# Autodesk Inventor assembly: turret_assembly
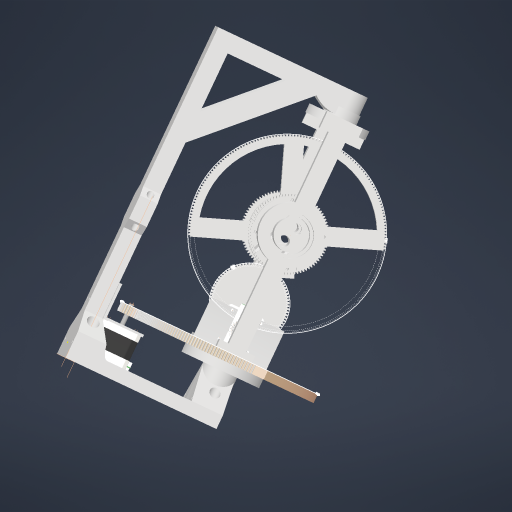
[picture p0: Inventor's stored thumbnail of the model, 512x512]
Saved by Autodesk Inventor 2023.2 (Build 272271000, 271)
## iProperties
Created: 2020-09-03
Part Number: turret_assembly
Document SubType Name: Assembly
Designer: bober
Author: bober
## Documents named in this file (19)
- F:\Turret\Our\Models\turret_assembly.iam
- F:\Turret\Our\Models\turret_assembly\Design Accelerator\vertical_axis_small_gear.ipt
- F:\Turret\Our\Models\turret_assembly\Design Accelerator\vertical_axis_bigl_gear.ipt
- F:\Turret\Our\Models\turret_assembly\Design Accelerator\horizontal_axis_big_gear.ipt
- F:\Turret\Our\Models\turret_assembly\Design Accelerator\pylon.ipt
- F:\Turret\Our\Models\turret_assembly\Design Accelerator\upper_grip.ipt
- F:\Turret\Our\Models\turret_assembly\Design Accelerator\main_stand_lower_half.ipt
- F:\Turret\Our\Models\turret_assembly\Design Accelerator\main_stand_upper_half.ipt
- F:\Turret\Our\Models\step_motor\Nema 17 Motor a Pasos 17HS4401.iam
- F:\Turret\Our\Models\turret_assembly\Design Accelerator\horizontal_lower_bearing_holder.ipt
- F:\Turret\Our\Models\turret_assembly\Design Accelerator\horizontal_axis_motor_metal_holder.ipt
- F:\Turret\Our\Models\turret_assembly\Design Accelerator\vertical_axis_motor_metal_holder.ipt
- F:\Turret\Our\Models\turret_assembly\Design Accelerator\Swash_distance.ipt
- F:\Turret\Our\Models\turret_assembly\Design Accelerator\big_actuator_holder.ipt
- F:\Turret\Our\Models\pylon_actuator_holder.ipt
- F:\Turret\Our\Models\pylon_actuator_holder_jaw.ipt
- F:\Turret\Our\Models\vertical_axis_hal_holder.ipt
- F:\Turret\Our\Models\turret_assembly\Design Accelerator\Spur Gears1.iam
- F:\Turret\Our\Models\turret_assembly\Design Accelerator\horizontal_axis_hal_gearr.ipt
## Components (23 placed, 18 different names)
1. vertical_axis_small_gear:1 — Tangent:1, Mate:4, Flush:1
2. horizontal_axis_big_gear:1 — Rigid:19, Insert:10
3. vertical_axis_small_gear:2 — Rotational:14
4. vertical_axis_bigl_gear:2 — Rigid:11, Rigid:12, Rigid:20, Rigid:21, Tangent:1, Flush:1
5. pylon:1 — Rigid:21, Flush:2, Insert:1
6. pylon:2 — Rigid:20, Rigid:22, Insert:4
7. upper_grip:1 — Rigid:22, Flush:3, Insert:11, Insert:12
8. main_stand_lower_half:1 — Rigid:5, Rotational:12, Mate:1, Mate:2, Rigid:15, Mate:3
9. main_stand_upper_half:1 — Rigid:15
10. Nema 17 Motor a Pasos 17HS4401:2 [sub-assembly] — Mate:3, Mate:4
11. Nema 17 Motor a Pasos 17HS4401:3 [sub-assembly] — Rigid:13, Rotational:14
12. horizontal_lower_bearing_holder:1 — Rigid:11, Rotational:11
13. horizontal_axis_motor_metal_holder:1 — Rigid:12, Rigid:13
14. vertical_axis_motor_metal_holder:1 — Rigid:5
15. Swash_distance:1 — Rotational:11, Rotational:12
16. big_actuator_holder:1 — Rigid:19, Insert:2, Insert:3
17. pylon_actuator_holder:1 — Flush:2, Insert:6, Insert:1, Insert:2, Insert:3, Insert:7, Flush:4, Flush:5, Mate:5
18. pylon_actuator_holder_jaw:1 — Insert:6, Insert:7
19. pylon_actuator_holder:2 — Insert:8, Insert:4, Insert:9, Insert:10
20. pylon_actuator_holder_jaw:2 — Insert:8, Insert:9
21. vertical_axis_hal_holder:1 — Flush:3, Insert:11, Insert:12
22. Spur Gears:1 [sub-assembly] — Flush:4
23. horizontal_axis_hal_gearr:1 — Flush:5, Mate:5
## Relationships (34: Insert 11, WeldJoint 9, Mate 5, Flush 5, RevoluteJoint 3, Tangent 1)
- Rigid:5 [WeldJoint]: main_stand_lower_half:1 ↔ vertical_axis_motor_metal_holder:1
- Rigid:11 [WeldJoint]: vertical_axis_bigl_gear:2 ↔ horizontal_lower_bearing_holder:1
- Rotational:11 [RevoluteJoint]: horizontal_lower_bearing_holder:1 ↔ Swash_distance:1
- Rotational:12 [RevoluteJoint]: main_stand_lower_half:1 ↔ Swash_distance:1
- Mate:1: main_stand_lower_half:1
- Mate:2: main_stand_lower_half:1
- Rigid:12 [WeldJoint]: vertical_axis_bigl_gear:2 ↔ horizontal_axis_motor_metal_holder:1
- Rigid:13 [WeldJoint]: Nema 17 Motor a Pasos 17HS4401:3 ↔ horizontal_axis_motor_metal_holder:1
- Rotational:14 [RevoluteJoint]: vertical_axis_small_gear:2 ↔ Nema 17 Motor a Pasos 17HS4401:3
- Rigid:15 [WeldJoint]: main_stand_lower_half:1 ↔ main_stand_upper_half:1
- Rigid:19 [WeldJoint]: horizontal_axis_big_gear:1 ↔ big_actuator_holder:1
- Rigid:20 [WeldJoint]: vertical_axis_bigl_gear:2 ↔ pylon:2
- Rigid:21 [WeldJoint]: vertical_axis_bigl_gear:2 ↔ pylon:1
- Rigid:22 [WeldJoint]: pylon:2 ↔ upper_grip:1
- Tangent:1: vertical_axis_small_gear:1 ↔ vertical_axis_bigl_gear:2
- Mate:3: main_stand_lower_half:1 ↔ Nema 17 Motor a Pasos 17HS4401:2
- Mate:4: vertical_axis_small_gear:1 ↔ Nema 17 Motor a Pasos 17HS4401:2
- Flush:1: vertical_axis_small_gear:1 ↔ vertical_axis_bigl_gear:2
- Flush:2: pylon:1 ↔ pylon_actuator_holder:1
- Insert:6: pylon_actuator_holder:1 ↔ pylon_actuator_holder_jaw:1
- Insert:1: pylon:1 ↔ pylon_actuator_holder:1
- Insert:2 (-97.5 mm): big_actuator_holder:1 ↔ pylon_actuator_holder:1
- Insert:3 (-97.5 mm): big_actuator_holder:1 ↔ pylon_actuator_holder:1
- Insert:8: pylon_actuator_holder:2 ↔ pylon_actuator_holder_jaw:2
- Insert:4: pylon:2 ↔ pylon_actuator_holder:2
- Insert:7: pylon_actuator_holder:1 ↔ pylon_actuator_holder_jaw:1
- Insert:9: pylon_actuator_holder:2 ↔ pylon_actuator_holder_jaw:2
- Insert:10 (-30.5 mm): horizontal_axis_big_gear:1 ↔ pylon_actuator_holder:2
- Flush:3: upper_grip:1 ↔ vertical_axis_hal_holder:1
- Flush:4: pylon_actuator_holder:1 ↔ Spur Gears:1
- Insert:11: upper_grip:1 ↔ vertical_axis_hal_holder:1
- Insert:12: upper_grip:1 ↔ vertical_axis_hal_holder:1
- Flush:5: pylon_actuator_holder:1 ↔ horizontal_axis_hal_gearr:1
- Mate:5 (80 mm): pylon_actuator_holder:1 ↔ horizontal_axis_hal_gearr:1
## Named parameters: d111_d107 = 0 mm
